(part 1 of 2)
# Autodesk Inventor assembly: #SHOOTER.3
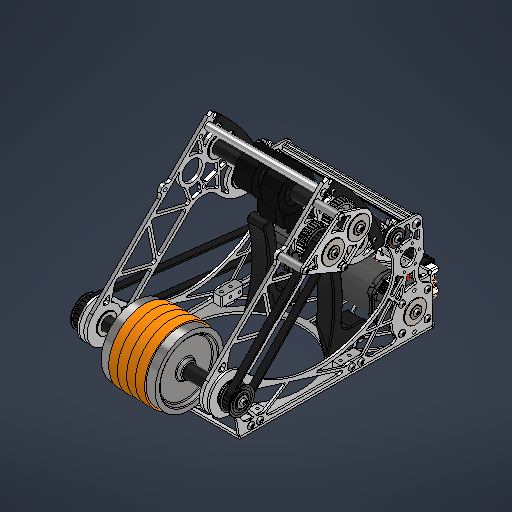
[picture p0: Inventor's stored thumbnail of the model, 512x512]
Saved by Autodesk Inventor 2026.1 (Build 301233020, 233B)
## iProperties
Created: 2026-01-27
Part Number: #SHOOTER.3
Document SubType Name: Assembly
Designer: Owen L
Mass: 4989.7 g
Surface Area: 9374.65 cm^2
Volume: 1663.66 cm^3
Density: 2.99923 g/cm^3
Author: Owen L
## Documents named in this file (57)
- C:\Users\Owen\Documents\GitHub\2026-Robot-Mechanical\Shooter\Shooter #3\#SHOOTER.3.iam
- C:\Users\Owen\Documents\GitHub\2026-Robot-Mechanical\Shooter\Shooter #3\PLATE,SHOOTER,SIDE.ipt
- C:\Users\Owen\Documents\GitHub\2026-Robot-Mechanical\#1_CAD Library\Electronics\CONTROLS,SPARK_FLEX.ipt
- C:\Users\Owen\Documents\GitHub\2026-Robot-Mechanical\#1_CAD Library\Electronics\CONTROLS,SPARK_MAX.ipt
- C:\Users\Owen\Documents\GitHub\2026-Robot-Mechanical\#1_CAD Library\Power Transmission\Bushings\PURCHASED,BUSHING,13.75mmID,0.75inOD.ipt
- C:\Users\Owen\Documents\GitHub\2026-Robot-Mechanical\#1_CAD Library\Power Transmission\Bearings\PURCHASED,HEX_BEARING.ipt
- C:\Users\Owen\Documents\GitHub\2026-Robot-Mechanical\#1_CAD Library\Motors\MOTOR,REV,NEO,VORTEX.ipt
- C:\Users\Owen\Documents\GitHub\2026-Robot-Mechanical\#1_CAD Library\Motors\MOTOR,REV,NEO,550.ipt
- C:\Users\Owen\Documents\GitHub\2026-Robot-Mechanical\#1_CAD Library\Power Transmission\UltraPlanetary\PURCHASED,REV,ULTRAPLANETARY,2-STAGE.iam
- C:\Users\Owen\Documents\GitHub\2026-Robot-Mechanical\Shooter\Shooter #3\#SHOOTER.3\Design Accelerator\PLATE,HOOD,SIDE.ipt
- C:\Users\Owen\Documents\GitHub\2026-Robot-Mechanical\Shooter\Shooter #3\#SHOOTER.3\Design Accelerator\PLATE.HOOD,PINION,GEAR.ipt
- C:\Users\Owen\Documents\GitHub\2026-Robot-Mechanical\Shooter\Shooter #3\STOCK,HEX,ROUND,HOOD.ipt
- C:\Users\Owen\Documents\GitHub\2026-Robot-Mechanical\#1_CAD Library\Power Transmission\Pulleys\PURCHASED,HTD5mm,20T,PULLEY.ipt
- C:\Users\Owen\Documents\GitHub\2026-Robot-Mechanical\Shooter\Shooter #3\STOCK,SHAFT,HEX,MOTORS.ipt
- C:\Users\Owen\Documents\GitHub\2026-Robot-Mechanical\Shooter\Shooter #3\#SHOOTER.3\Design Accelerator\PLATE,HOOD,DRIVE,GEAR,SHAFT.ipt
- C:\Users\Owen\Documents\GitHub\2026-Robot-Mechanical\Shooter\Shooter #3\#SHOOTER.3\Design Accelerator\PLATE,HOOD,DRIVE,GEAR,MOTOR.ipt
- C:\Users\Owen\Documents\GitHub\2026-Robot-Mechanical\#1_CAD Library\Power Transmission\Pulleys\PURCHASED,HTD5mm,24T,PULLEY.ipt
- C:\Users\Owen\Documents\GitHub\2026-Robot-Mechanical\Shooter\Shooter #3\STOCK,SHAFT,HEX,SHOOTER.ipt
- C:\Users\Owen\Documents\GitHub\2026-Robot-Mechanical\Shooter\Shooter #3\#SHOOTER.3\PURCHASED,10-32,0.375inOD,STANDOFF.ipt
- C:\Users\Owen\Documents\GitHub\2026-Robot-Mechanical\Shooter\Shooter #3\PLATE,BEARING,MOUNT.ipt
- C:\Users\Owen\Documents\GitHub\2026-Robot-Mechanical\Shooter\Shooter #3\STOCK,SHAFT,HEX,HOOD,WHEELS,LONG.ipt
- C:\Users\Owen\Documents\GitHub\2026-Robot-Mechanical\Shooter\Shooter #3\STOCK,SHAFT,HEX,HOOD,REVERSER.ipt
- C:\Users\Owen\Documents\GitHub\2026-Robot-Mechanical\Shooter\Shooter #3\STOCK,SHAFT,HEX,HOOD,WHEELS,SHORT.ipt
- C:\Users\Owen\Documents\GitHub\2026-Robot-Mechanical\Shooter\Shooter #3\PLATE,SHOOTER,BOTTOM.ipt
- C:\Users\Owen\Documents\GitHub\2026-Robot-Mechanical\Shooter\Shooter #3\PLATE,SHOOTER,BACK.ipt
- C:\Users\Owen\Documents\GitHub\2026-Robot-Mechanical\Shooter\Shooter #3\STOCK,CHURRO,HEX,BACK.ipt
- C:\Users\Owen\Documents\GitHub\2026-Robot-Mechanical\Shooter\Shooter #3\PURCHASED,WASHER.ipt
- C:\Users\Owen\Documents\GitHub\2026-Robot-Mechanical\#1_CAD Library\Wheels\Shooter\PURCHASED,2inOD,HEX,SHOOTER,WHEEL.ipt
- C:\Users\Owen\Documents\GitHub\2026-Robot-Mechanical\#1_CAD Library\Building Materials\Fasteners\Bolts\PURCHASED,0.25-20x0.5in,BUTTONHEAD,BOLT.ipt
- C:\Users\Owen\Documents\GitHub\2026-Robot-Mechanical\#1_CAD Library\Building Materials\Fasteners\Bolts\PURCHASED,10-32x0.5in,BUTTONHEAD,BOLT.ipt
- C:\Users\Owen\Documents\GitHub\2026-Robot-Mechanical\#1_CAD Library\Building Materials\Fasteners\Bolts\PURCHASED,M3x10mm,BUTTONHEAD,BOLT.ipt
- C:\Users\Owen\Documents\GitHub\2026-Robot-Mechanical\#1_CAD Library\Wheels\Shooter\PURCHASED,4inOD,HEX,SHOOTER,WHEEL.ipt
- C:\Users\Owen\Documents\GitHub\2026-Robot-Mechanical\Shooter\Shooter #3\3DPRINT,HOOD,DRIVEGEAR,SPACER.ipt
- C:\Users\Owen\Documents\GitHub\2026-Robot-Mechanical\Shooter\Shooter #3\3DPRINT,REVERSERGEAR,SPACER.ipt
- C:\Users\Owen\Documents\GitHub\2026-Robot-Mechanical\Shooter\Shooter #3\3DPRINT,BACKROLLERS,OPENSIDE,SPACER.ipt
- C:\Users\Owen\Documents\GitHub\2026-Robot-Mechanical\Shooter\Shooter #3\3DPRINT,BACKROLLERS,PULLEYSIDE,SPACER.ipt
- C:\Users\Owen\Documents\GitHub\2026-Robot-Mechanical\Shooter\Shooter #3\3DPRINT,BACKROLLERS,INTERROLLER,SPACER.ipt
- C:\Users\Owen\Documents\GitHub\2026-Robot-Mechanical\Shooter\Shooter #3\PLATE,FLYWHEEL.ipt
- C:\Users\Owen\Documents\GitHub\2026-Robot-Mechanical\Shooter\Shooter #3\3DPRINT,FLYWHEEL,SPACER.ipt
- C:\Users\Owen\Documents\GitHub\2026-Robot-Mechanical\#1_CAD Library\Power Transmission\Gears\PURCHASED,GEAR,20DP,30T,HEX.ipt
- C:\Users\Owen\Documents\GitHub\2026-Robot-Mechanical\Shooter\Shooter #3\3DPRINT,BACKRAIL.ipt
- C:\Users\Owen\Documents\GitHub\2026-Robot-Mechanical\Shooter\Shooter #3\3DPRINT,BACKRAIL_MIR.ipt
- C:\Users\Owen\Documents\GitHub\2026-Robot-Mechanical\Shooter\Shooter #3\PLATE,NUTBLOCK.ipt
- C:\Users\Owen\Documents\GitHub\2026-Robot-Mechanical\Shooter\Shooter #3\3DPRINT,SPARK_MAX,MOUNT.ipt
- C:\Users\Owen\Documents\GitHub\2026-Robot-Mechanical\#1_CAD Library\Building Materials\Fasteners\Bolts\PURCHASED,M4x12mm,BUTTONHEAD,BOLT.ipt
- C:\Users\Owen\Documents\GitHub\2026-Robot-Mechanical\Shooter\Shooter #3\STANDIN,130T,HTD5mm,BELT.ipt
- C:\Users\Owen\Documents\GitHub\2026-Robot-Mechanical\Shooter\Shooter #3\STANDIN,45T,HTD5mm,BELT.ipt
- C:\Users\Owen\Documents\GitHub\2026-Robot-Mechanical\Shooter\Shooter #3\STANDIN,90T,HTD5mm,BELT.ipt
- C:\Users\Owen\Documents\GitHub\2026-Robot-Mechanical\Shooter\Shooter #3\3DPRINT,FLYWHEELTOHOOD,SPACER.ipt
- C:\Users\Owen\Documents\GitHub\2026-Robot-Mechanical\Shooter\Shooter #3\STOCK,HOOD,SPACER,10-32,6.25in.ipt
- C:\Users\Owen\Documents\GitHub\2026-Robot-Mechanical\Shooter\Shooter #3\3DPRINT,SIDEPLATETOHOOD,SPACER .ipt
- C:\Users\Owen\Documents\GitHub\2026-Robot-Mechanical\Shooter\Shooter #3\3DPRINT,SIDEPLATETOHOODGEAR,SPACER.ipt
- C:\Users\Owen\Documents\GitHub\2026-Robot-Mechanical\Shooter\Shooter #3\3DPRINT,BUSHINGTOHOODDRIVEGEAR,SPACER.ipt
- C:\Users\Owen\Documents\GitHub\2026-Robot-Mechanical\Shooter\Shooter #3\PLATE,NUTBLOCK,BACK.ipt
- C:\Users\Owen\Documents\GitHub\2026-Robot-Mechanical\Shooter\Shooter #3\3DPRINT,HOOD,ALIGNMENT,PLATES.ipt
- C:\Users\Owen\Documents\GitHub\2026-Robot-Mechanical\#1_CAD Library\Building Materials\Fasteners\Bolts\PURCHASED,M3x16mm,BUTTONHEAD,BOLT.ipt
- C:\Users\Owen\Documents\GitHub\2026-Robot-Mechanical\#1_CAD Library\Building Materials\Fasteners\Nuts\PURCHASED,M3,NYLOCK,NUT.ipt
## Components (193 placed, 56 different names)
1. PLATE,SHOOTER,SIDE:1 — Insert:2, Mate:2, Insert:3, Insert:4, Mate:6, Mate:36, Insert:39, Insert:57, Insert:58, Insert:59, Insert:60, Insert:82, Insert:83, Insert:84, Insert:85, Mate:120, Insert:108, Insert:110, Insert:111, Insert:112, Insert:113, Insert:114, Insert:146, Mate:138, Mate:139
2. CONTROLS,SPARK_FLEX:1 — Mate:3, Mate:4, Mate:5, Insert:36, Insert:37
3. CONTROLS,SPARK_FLEX:2 — Mate:12, Mate:13, Mate:14, Insert:34, Insert:35
4. CONTROLS,SPARK_MAX:1 — Mate:75, Mate:135, Mate:136
5. PURCHASED,BUSHING,13.75mmID,0.75inOD:1 — Insert:3, Mate:8, Mate:166, Mate:173
6. PURCHASED,BUSHING,13.75mmID,0.75inOD:2 — Insert:7, Mate:11, Mate:170
7. PURCHASED,HEX_BEARING:1 — Insert:4, Mate:30, Mate:31, Mate:46, Mate:156
8. MOTOR,REV,NEO,VORTEX:1 — Mate:3, Mate:4, Mate:5
9. MOTOR,REV,NEO,VORTEX:2 — Mate:12, Mate:13, Mate:14
10. MOTOR,REV,NEO,550:1 — Insert:1, Mate:1
11. PURCHASED,REV,ULTRAPLANETARY,2-STAGE:1 [sub-assembly] — Insert:1, Mate:1, Insert:2, Mate:2, Flush:1, Insert:14, Mate:26
12. PLATE,HOOD,SIDE:1 — Mate:6, Mate:7, Mate:15, Insert:15, Insert:16, Mate:27, Insert:20, Mate:81, Mate:82, Symmetry:1, Insert:152, Insert:154, Insert:155, Mate:174, Insert:161, Insert:163, Insert:164, Insert:165
13. PLATE.HOOD,PINION,GEAR:1 — Mate:22, Mate:23, Mate:163, Mate:167
14. PLATE,HOOD,SIDE:2 — Mate:7, Mate:15, Insert:17, Insert:18, Mate:27, Insert:21, Insert:24, Insert:25, Insert:26, Insert:31, Insert:91, Insert:92, Insert:93, Symmetry:1, Mate:147, Mate:148, Mate:150, Insert:153, Insert:156, Insert:157, Insert:166, Insert:167, Insert:168, Insert:169
15. STOCK,HEX,ROUND,HOOD:1 — Mate:8, Flush:1, Mate:11, Mate:20, Mate:21, Mate:22, Mate:23, Mate:24, Mate:25, Insert:47, Insert:55, Mate:83, Mate:84, Mate:164, Mate:165, Mate:168, Mate:169, Mate:171, Mate:172
16. PURCHASED,HTD5mm,20T,PULLEY:1 — Mate:59, Mate:60, Mate:64, Mate:97, Mate:152
17. PLATE,SHOOTER,SIDE:2 — Insert:7, Insert:19, Mate:36, Insert:32, Insert:33, Insert:38, Insert:40, Insert:73, Insert:74, Insert:75, Insert:76, Insert:101, Insert:104, Insert:124, Insert:125, Insert:126, Insert:127, Insert:145, Mate:149
18. PURCHASED,HEX_BEARING:3 — Mate:18, Mate:19, Mate:47, Insert:39
19. PURCHASED,HEX_BEARING:4 — Insert:38
20. PLATE.HOOD,PINION,GEAR:2 — Mate:20, Mate:21, Mate:85
21. STOCK,SHAFT,HEX,MOTORS:1 — Mate:18, Mate:19, Mate:28, Mate:29, Flush:6, Insert:42, Insert:56, Rotation:1
22. PLATE,HOOD,DRIVE,GEAR,SHAFT:1 — Mate:24, Mate:25, Flush:2
23. PLATE,HOOD,DRIVE,GEAR,MOTOR:1 — Insert:14, Mate:26, Flush:2, Insert:77, Insert:78, Insert:79, Insert:80, Insert:81
24. PURCHASED,HEX_BEARING:5 — Insert:15, Mate:37, Mate:38, Flush:3
25. PURCHASED,HEX_BEARING:6 — Insert:16, Mate:39, Mate:40, Flush:4
26. PURCHASED,HEX_BEARING:7 — Insert:17, Mate:64, Mate:128
27. PURCHASED,HEX_BEARING:8 — Insert:18, Mate:63
28. PURCHASED,HTD5mm,24T,PULLEY:1 — Mate:28, Mate:29, Mate:47, Flush:6, Mate:140
29. PURCHASED,HTD5mm,24T,PULLEY:2 — Mate:32, Mate:33, Mate:46, Flush:7
30. STOCK,SHAFT,HEX,SHOOTER:1 — Mate:30, Mate:31, Mate:32, Mate:33, Flush:7, Insert:50, Insert:51, Mate:76, Mate:77, Mate:79, Mate:80, Mate:107, Mate:108, Mate:110, Mate:111, Mate:113, Mate:114, Mate:116, Mate:117, Mate:141, Mate:142, Rotation:1, Flush:9, Mate:153, Mate:154, Mate:157, Mate:158, Mate:160, Mate:161
31. PURCHASED,HEX_BEARING:9 — Insert:19, Mate:155
32. PURCHASED,HEX_BEARING:10 — Insert:20, Mate:156, Mate:162
33. PURCHASED,HEX_BEARING:11 — Insert:21, Mate:115, Mate:159
34. PURCHASED,HEX_BEARING:12 — Insert:31, Mate:41, Mate:42, Flush:5, Mate:129
35. PURCHASED,10-32,0.375inOD,STANDOFF:1 — Insert:24, Insert:97
36. PURCHASED,10-32,0.375inOD,STANDOFF:2 — Insert:25
37. PURCHASED,10-32,0.375inOD,STANDOFF:3 — Insert:26
38. PLATE,BEARING,MOUNT:1 — Insert:94, Insert:96, Insert:97, Insert:98, Insert:99, Insert:100
39. PURCHASED,HEX_BEARING:14 — Mate:88, Mate:121, Mate:122, Insert:96
40. PURCHASED,HEX_BEARING:15 — Insert:94, Mate:123
41. STOCK,SHAFT,HEX,HOOD,WHEELS,LONG:1 — Mate:37, Mate:38, Flush:3, Mate:59, Mate:60, Insert:48, Insert:53, Mate:65, Mate:66, Mate:67, Mate:68, Mate:86, Mate:87, Mate:89, Mate:90, Mate:95, Mate:96, Mate:101, Mate:102, Mate:121, Mate:122, Mate:126, Mate:127
42. STOCK,SHAFT,HEX,HOOD,REVERSER:1 — Mate:41, Mate:42, Flush:5, Insert:52, Insert:86, Mate:123, Mate:124, Mate:125, Mate:144, Mate:145
43. STOCK,SHAFT,HEX,HOOD,WHEELS,SHORT:1 — Mate:39, Mate:40, Flush:4, Mate:61, Mate:62, Insert:49, Insert:54, Mate:69, Mate:70, Mate:71, Mate:72, Mate:92, Mate:93, Mate:98, Mate:99, Mate:104, Mate:105
44. PLATE,SHOOTER,BOTTOM:1 — Mate:120, Mate:131, Insert:102, Insert:103, Insert:107, Insert:109, Insert:115, Insert:116, Insert:117, Insert:118, Insert:119, Insert:120, Insert:121, Insert:122, Insert:123, Insert:137, Insert:138, Insert:139, Insert:140, Insert:141, Insert:142, Insert:143, Insert:144, Insert:151, Mate:137, Insert:158, Mate:174, Insert:160
45. PLATE,SHOOTER,BACK:1 — Insert:32, Insert:33, Insert:34, Insert:35, Insert:36, Insert:37, Mate:75, Insert:128, Insert:129, Insert:133, Mate:134, Insert:159
46. PURCHASED,HTD5mm,20T,PULLEY:2 — Mate:61, Mate:62, Mate:63, Mate:100
47. STOCK,CHURRO,HEX,BACK:1 — Insert:40
48. PURCHASED,WASHER:1 — Insert:42, Insert:61
49. PURCHASED,2inOD,HEX,SHOOTER,WHEEL:1 — Mate:65, Mate:66, Mate:73, Mate:103
50. PURCHASED,2inOD,HEX,SHOOTER,WHEEL:2 — Mate:67, Mate:68, Mate:73, Mate:82, Flush:8, Mate:91
51. PURCHASED,2inOD,HEX,SHOOTER,WHEEL:3 — Mate:69, Mate:70, Mate:74, Mate:106
52. PURCHASED,2inOD,HEX,SHOOTER,WHEEL:4 — Mate:71, Mate:72, Mate:74, Flush:8, Mate:94
53. PURCHASED,0.25-20x0.5in,BUTTONHEAD,BOLT:1 — Insert:146
54. PURCHASED,0.25-20x0.5in,BUTTONHEAD,BOLT:4 — Insert:145
55. PURCHASED,10-32x0.5in,BUTTONHEAD,BOLT:1 — Insert:57
56. PURCHASED,M3x10mm,BUTTONHEAD,BOLT:1 — Insert:77
57. PURCHASED,WASHER:2 — Insert:47, Insert:62
58. PURCHASED,WASHER:3 — Insert:48, Insert:64
59. PURCHASED,WASHER:4 — Insert:49, Insert:63
60. PURCHASED,WASHER:5 — Insert:50, Insert:65
61. PURCHASED,WASHER:6 — Insert:51, Insert:66
62. PURCHASED,WASHER:7 — Insert:52, Insert:67
63. PURCHASED,WASHER:8 — Insert:53, Insert:68
64. PURCHASED,WASHER:9 — Insert:54, Insert:69
65. PURCHASED,WASHER:10 — Insert:55, Insert:70
66. PURCHASED,WASHER:11 — Insert:56, Insert:71
67. PURCHASED,10-32x0.5in,BUTTONHEAD,BOLT:2 — Insert:60
68. PURCHASED,10-32x0.5in,BUTTONHEAD,BOLT:3 — Insert:58
69. PURCHASED,10-32x0.5in,BUTTONHEAD,BOLT:4 — Insert:59
70. PURCHASED,10-32x0.5in,BUTTONHEAD,BOLT:5 — Insert:61
71. PURCHASED,10-32x0.5in,BUTTONHEAD,BOLT:6 — Insert:62
72. PURCHASED,10-32x0.5in,BUTTONHEAD,BOLT:7 — Insert:63
73. PURCHASED,10-32x0.5in,BUTTONHEAD,BOLT:8 — Insert:65
74. PURCHASED,10-32x0.5in,BUTTONHEAD,BOLT:9 — Insert:64
75. PURCHASED,10-32x0.5in,BUTTONHEAD,BOLT:10 — Insert:66
76. PURCHASED,10-32x0.5in,BUTTONHEAD,BOLT:11 — Insert:67
77. PURCHASED,10-32x0.5in,BUTTONHEAD,BOLT:12 — Insert:68
78. PURCHASED,10-32x0.5in,BUTTONHEAD,BOLT:13 — Insert:69
79. PURCHASED,10-32x0.5in,BUTTONHEAD,BOLT:14 — Insert:70
80. PURCHASED,10-32x0.5in,BUTTONHEAD,BOLT:15 — Insert:71
81. PURCHASED,10-32x0.5in,BUTTONHEAD,BOLT:16 — Insert:87
82. PURCHASED,10-32x0.5in,BUTTONHEAD,BOLT:17 — Insert:73
83. PURCHASED,10-32x0.5in,BUTTONHEAD,BOLT:18 — Insert:74
84. PURCHASED,10-32x0.5in,BUTTONHEAD,BOLT:19 — Insert:75
85. PURCHASED,10-32x0.5in,BUTTONHEAD,BOLT:20 — Insert:76
86. PURCHASED,M3x10mm,BUTTONHEAD,BOLT:2 — Insert:78
87. PURCHASED,M3x10mm,BUTTONHEAD,BOLT:3 — Insert:80
88. PURCHASED,M3x10mm,BUTTONHEAD,BOLT:4 — Insert:79
89. PURCHASED,M3x10mm,BUTTONHEAD,BOLT:5 — Insert:81
90. PURCHASED,M3x10mm,BUTTONHEAD,BOLT:6 — Insert:82
91. PURCHASED,M3x10mm,BUTTONHEAD,BOLT:7 — Insert:83
92. PURCHASED,M3x10mm,BUTTONHEAD,BOLT:8 — Insert:84
93. PURCHASED,M3x10mm,BUTTONHEAD,BOLT:9 — Insert:85
94. PURCHASED,4inOD,HEX,SHOOTER,WHEEL:1 — Mate:76, Mate:77, Mate:78, Mate:112
95. PURCHASED,4inOD,HEX,SHOOTER,WHEEL:2 — Mate:78, Mate:79, Mate:80, Mate:81, Mate:109
96. 3DPRINT,HOOD,DRIVEGEAR,SPACER:1 — Mate:83, Mate:84, Mate:85, Mate:163
97. 3DPRINT,REVERSERGEAR,SPACER:1 — Mate:86, Mate:87, Mate:88
98. 3DPRINT,BACKROLLERS,OPENSIDE,SPACER:1 — Mate:89, Mate:90, Mate:91
99. 3DPRINT,BACKROLLERS,OPENSIDE,SPACER:2 — Mate:92, Mate:93, Mate:94
100. 3DPRINT,BACKROLLERS,PULLEYSIDE,SPACER:1 — Mate:95, Mate:96, Mate:97
101. 3DPRINT,BACKROLLERS,PULLEYSIDE,SPACER:2 — Mate:98, Mate:99, Mate:100
102. 3DPRINT,BACKROLLERS,INTERROLLER,SPACER:1 — Mate:101, Mate:102, Mate:103
103. 3DPRINT,BACKROLLERS,INTERROLLER,SPACER:2 — Mate:104, Mate:105, Mate:106
104. PLATE,FLYWHEEL:1 — Mate:107, Mate:108, Mate:109, Mate:118, Mate:132
105. PLATE,FLYWHEEL:2 — Mate:110, Mate:111, Mate:112
106. 3DPRINT,FLYWHEEL,SPACER:1 — Mate:113, Mate:114, Mate:115
107. 3DPRINT,FLYWHEEL,SPACER:2 — Mate:116, Mate:117, Mate:118
108. PURCHASED,WASHER:12 — Insert:86, Insert:87
109. PURCHASED,10-32x0.5in,BUTTONHEAD,BOLT:21 — Insert:99
110. PURCHASED,10-32x0.5in,BUTTONHEAD,BOLT:22 — Insert:98
111. PURCHASED,10-32x0.5in,BUTTONHEAD,BOLT:23 — Insert:100
112. PURCHASED,10-32x0.5in,BUTTONHEAD,BOLT:24 — Insert:91
113. PURCHASED,10-32x0.5in,BUTTONHEAD,BOLT:25 — Insert:92
114. PURCHASED,10-32x0.5in,BUTTONHEAD,BOLT:26 — Insert:93
115. PURCHASED,GEAR,20DP,30T,HEX:1 — Mate:124, Mate:125, Mate:129, Mate:146
116. PURCHASED,GEAR,20DP,30T,HEX:2 — Mate:126, Mate:127, Mate:128
117. 3DPRINT,BACKRAIL:1 — Mate:131, Mate:132, Insert:158
118. 3DPRINT,BACKRAIL_MIR:1 — Insert:151, Mate:137
119. PLATE,NUTBLOCK:1 — Insert:101, Insert:102
120. PLATE,NUTBLOCK:2 — Insert:103, Insert:104
121. PLATE,NUTBLOCK:4 — Insert:107, Insert:108
122. PLATE,NUTBLOCK:5 — Insert:109, Insert:110
123. PURCHASED,10-32x0.5in,BUTTONHEAD,BOLT:27 — Insert:114
124. PURCHASED,10-32x0.5in,BUTTONHEAD,BOLT:28 — Insert:113
125. PURCHASED,10-32x0.5in,BUTTONHEAD,BOLT:29 — Insert:112
126. PURCHASED,10-32x0.5in,BUTTONHEAD,BOLT:30 — Insert:111
127. PURCHASED,10-32x0.5in,BUTTONHEAD,BOLT:31 — Insert:115
128. PURCHASED,10-32x0.5in,BUTTONHEAD,BOLT:32 — Insert:116
129. PURCHASED,10-32x0.5in,BUTTONHEAD,BOLT:33 — Insert:117
130. PURCHASED,10-32x0.5in,BUTTONHEAD,BOLT:34 — Insert:118
131. PURCHASED,10-32x0.5in,BUTTONHEAD,BOLT:35 — Insert:119
132. PURCHASED,10-32x0.5in,BUTTONHEAD,BOLT:36 — Insert:120
133. PURCHASED,10-32x0.5in,BUTTONHEAD,BOLT:37 — Insert:121
134. PURCHASED,10-32x0.5in,BUTTONHEAD,BOLT:38 — Insert:122
135. PURCHASED,10-32x0.5in,BUTTONHEAD,BOLT:39 — Insert:123
136. PURCHASED,10-32x0.5in,BUTTONHEAD,BOLT:40 — Insert:124
137. PURCHASED,10-32x0.5in,BUTTONHEAD,BOLT:41 — Insert:125
138. PURCHASED,10-32x0.5in,BUTTONHEAD,BOLT:42 — Insert:126
139. PURCHASED,10-32x0.5in,BUTTONHEAD,BOLT:43 — Insert:127
140. PURCHASED,10-32x0.5in,BUTTONHEAD,BOLT:44 — Insert:128
141. PURCHASED,10-32x0.5in,BUTTONHEAD,BOLT:45 — Insert:129
142. 3DPRINT,SPARK_MAX,MOUNT:1 — Insert:133, Mate:134, Mate:135, Mate:136, Insert:134, Insert:135, Insert:136
143. PURCHASED,10-32x0.5in,BUTTONHEAD,BOLT:46 — Insert:134
144. PURCHASED,10-32x0.5in,BUTTONHEAD,BOLT:47 — Insert:135
145. PURCHASED,10-32x0.5in,BUTTONHEAD,BOLT:48 — Insert:136
146. PURCHASED,M4x12mm,BUTTONHEAD,BOLT:1 — Insert:137
147. PURCHASED,M4x12mm,BUTTONHEAD,BOLT:2 — Insert:138
148. PURCHASED,M4x12mm,BUTTONHEAD,BOLT:3 — Insert:139
149. PURCHASED,M4x12mm,BUTTONHEAD,BOLT:4 — Insert:140
150. PURCHASED,M4x12mm,BUTTONHEAD,BOLT:5 — Insert:141
151. PURCHASED,M4x12mm,BUTTONHEAD,BOLT:6 — Insert:142
152. PURCHASED,M4x12mm,BUTTONHEAD,BOLT:7 — Insert:143
153. PURCHASED,M4x12mm,BUTTONHEAD,BOLT:8 — Insert:144
154. STANDIN,130T,HTD5mm,BELT:1 — Mate:138, Mate:139, Mate:140
155. PURCHASED,HTD5mm,20T,PULLEY:3 — Mate:141, Mate:142, Flush:9
156. PURCHASED,HTD5mm,20T,PULLEY:4 — Mate:144, Mate:145, Mate:146, Mate:151
157. STANDIN,45T,HTD5mm,BELT:1 — Mate:147, Mate:148, Mate:152
158. STANDIN,90T,HTD5mm,BELT:1 — Mate:149, Mate:150, Mate:151
159. 3DPRINT,FLYWHEELTOHOOD,SPACER:1 — Mate:153, Mate:154, Mate:155
160. STOCK,HOOD,SPACER,10-32,6.25in:1 — Insert:152
161. STOCK,HOOD,SPACER,10-32,6.25in:2 — Insert:153
162. PURCHASED,10-32x0.5in,BUTTONHEAD,BOLT:49 — Insert:154
163. PURCHASED,10-32x0.5in,BUTTONHEAD,BOLT:50 — Insert:156
164. PURCHASED,10-32x0.5in,BUTTONHEAD,BOLT:51 — Insert:155
165. PURCHASED,10-32x0.5in,BUTTONHEAD,BOLT:52 — Insert:157
166. 3DPRINT,SIDEPLATETOHOOD,SPACER :1 — Mate:157, Mate:158, Mate:159
167. 3DPRINT,SIDEPLATETOHOODGEAR,SPACER:1 — Mate:171, Mate:172, Mate:173
168. 3DPRINT,BUSHINGTOHOODDRIVEGEAR,SPACER:1 — Mate:164, Mate:165, Mate:166, Mate:167
169. 3DPRINT,SIDEPLATETOHOOD,SPACER :2 — Mate:160, Mate:161, Mate:162
170. 3DPRINT,BUSHINGTOHOODDRIVEGEAR,SPACER:2 — Mate:168, Mate:169, Mate:170
171. PLATE,NUTBLOCK,BACK:1 — Insert:159, Insert:160
172. 3DPRINT,HOOD,ALIGNMENT,PLATES:1 — Insert:161, Insert:165, Insert:174, Insert:175, Insert:176, Insert:177, Insert:178
173. 3DPRINT,HOOD,ALIGNMENT,PLATES:2 — Insert:163, Insert:164, Insert:179, Insert:180, Insert:181, Insert:182, Insert:183
174. 3DPRINT,HOOD,ALIGNMENT,PLATES:3 — Insert:166, Insert:167, Insert:170, Insert:171, Insert:172, Insert:173
175. 3DPRINT,HOOD,ALIGNMENT,PLATES:4 — Insert:168, Insert:169, Insert:184, Insert:185, Insert:186, Insert:187
176. PURCHASED,M3x16mm,BUTTONHEAD,BOLT:1 — Insert:170
177. PURCHASED,M3x16mm,BUTTONHEAD,BOLT:2 — Insert:171
178. PURCHASED,M3x16mm,BUTTONHEAD,BOLT:3 — Insert:172
179. PURCHASED,M3x16mm,BUTTONHEAD,BOLT:4 — Insert:173
180. PURCHASED,M3x16mm,BUTTONHEAD,BOLT:5 — Insert:174
181. PURCHASED,M3x16mm,BUTTONHEAD,BOLT:6 — Insert:175
182. PURCHASED,M3x16mm,BUTTONHEAD,BOLT:7 — Insert:176
183. PURCHASED,M3x16mm,BUTTONHEAD,BOLT:8 — Insert:177
184. PURCHASED,M3x16mm,BUTTONHEAD,BOLT:9 — Insert:178
185. PURCHASED,M3,NYLOCK,NUT:1 — Insert:186
186. PURCHASED,M3,NYLOCK,NUT:3 — Insert:187
187. PURCHASED,M3,NYLOCK,NUT:5 — Insert:185
188. PURCHASED,M3,NYLOCK,NUT:6 — Insert:184
189. PURCHASED,M3,NYLOCK,NUT:7 — Insert:183
190. PURCHASED,M3,NYLOCK,NUT:8 — Insert:182
191. PURCHASED,M3,NYLOCK,NUT:9 — Insert:181
192. PURCHASED,M3,NYLOCK,NUT:10 — Insert:180
193. PURCHASED,M3,NYLOCK,NUT:11 — Insert:179
## Relationships (314: Insert 153, Mate 150, Flush 9, Symmetry 1, RelateRotation 1)
- Insert:1: MOTOR,REV,NEO,550:1 ↔ PURCHASED,REV,ULTRAPLANETARY,2-STAGE:1
- Mate:1: MOTOR,REV,NEO,550:1 ↔ PURCHASED,REV,ULTRAPLANETARY,2-STAGE:1
- Insert:2: PLATE,SHOOTER,SIDE:1 ↔ PURCHASED,REV,ULTRAPLANETARY,2-STAGE:1
- Mate:2: PLATE,SHOOTER,SIDE:1 ↔ PURCHASED,REV,ULTRAPLANETARY,2-STAGE:1
- Insert:3: PLATE,SHOOTER,SIDE:1 ↔ PURCHASED,BUSHING,13.75mmID,0.75inOD:1
- Insert:4: PLATE,SHOOTER,SIDE:1 ↔ PURCHASED,HEX_BEARING:1
- Mate:3: CONTROLS,SPARK_FLEX:1 ↔ MOTOR,REV,NEO,VORTEX:1
- Mate:4: CONTROLS,SPARK_FLEX:1 ↔ MOTOR,REV,NEO,VORTEX:1
- Mate:5: CONTROLS,SPARK_FLEX:1 ↔ MOTOR,REV,NEO,VORTEX:1
- Mate:6: PLATE,SHOOTER,SIDE:1 ↔ PLATE,HOOD,SIDE:1
- Mate:7 (158.75 mm): PLATE,HOOD,SIDE:1 ↔ PLATE,HOOD,SIDE:2
- Mate:8: PURCHASED,BUSHING,13.75mmID,0.75inOD:1 ↔ STOCK,HEX,ROUND,HOOD:1
- Flush:1 (-6.35 mm): PURCHASED,REV,ULTRAPLANETARY,2-STAGE:1 ↔ STOCK,HEX,ROUND,HOOD:1
- Insert:7: PURCHASED,BUSHING,13.75mmID,0.75inOD:2 ↔ PLATE,SHOOTER,SIDE:2
- Mate:11: PURCHASED,BUSHING,13.75mmID,0.75inOD:2 ↔ STOCK,HEX,ROUND,HOOD:1
- Mate:12: CONTROLS,SPARK_FLEX:2 ↔ MOTOR,REV,NEO,VORTEX:2
- Mate:13: CONTROLS,SPARK_FLEX:2 ↔ MOTOR,REV,NEO,VORTEX:2
- Mate:14: CONTROLS,SPARK_FLEX:2 ↔ MOTOR,REV,NEO,VORTEX:2
- Mate:15: PLATE,HOOD,SIDE:1 ↔ PLATE,HOOD,SIDE:2
- Mate:18: PURCHASED,HEX_BEARING:3 ↔ STOCK,SHAFT,HEX,MOTORS:1
- Mate:19: PURCHASED,HEX_BEARING:3 ↔ STOCK,SHAFT,HEX,MOTORS:1
- Mate:20: STOCK,HEX,ROUND,HOOD:1 ↔ PLATE.HOOD,PINION,GEAR:2
- Mate:21: STOCK,HEX,ROUND,HOOD:1 ↔ PLATE.HOOD,PINION,GEAR:2
- Mate:22: PLATE.HOOD,PINION,GEAR:1 ↔ STOCK,HEX,ROUND,HOOD:1
- Mate:23: PLATE.HOOD,PINION,GEAR:1 ↔ STOCK,HEX,ROUND,HOOD:1
- Mate:24: STOCK,HEX,ROUND,HOOD:1 ↔ PLATE,HOOD,DRIVE,GEAR,SHAFT:1
- Mate:25: STOCK,HEX,ROUND,HOOD:1 ↔ PLATE,HOOD,DRIVE,GEAR,SHAFT:1
- Insert:14: PURCHASED,REV,ULTRAPLANETARY,2-STAGE:1 ↔ PLATE,HOOD,DRIVE,GEAR,MOTOR:1
- Mate:26: PURCHASED,REV,ULTRAPLANETARY,2-STAGE:1 ↔ PLATE,HOOD,DRIVE,GEAR,MOTOR:1
- Flush:2: PLATE,HOOD,DRIVE,GEAR,SHAFT:1 ↔ PLATE,HOOD,DRIVE,GEAR,MOTOR:1
- Insert:15: PLATE,HOOD,SIDE:1 ↔ PURCHASED,HEX_BEARING:5
- Insert:16: PLATE,HOOD,SIDE:1 ↔ PURCHASED,HEX_BEARING:6
- Insert:17: PLATE,HOOD,SIDE:2 ↔ PURCHASED,HEX_BEARING:7
- Insert:18: PLATE,HOOD,SIDE:2 ↔ PURCHASED,HEX_BEARING:8
- Mate:27: PLATE,HOOD,SIDE:1 ↔ PLATE,HOOD,SIDE:2
- Mate:28: STOCK,SHAFT,HEX,MOTORS:1 ↔ PURCHASED,HTD5mm,24T,PULLEY:1
- Mate:29: STOCK,SHAFT,HEX,MOTORS:1 ↔ PURCHASED,HTD5mm,24T,PULLEY:1
- Mate:30: PURCHASED,HEX_BEARING:1 ↔ STOCK,SHAFT,HEX,SHOOTER:1
- Mate:31: PURCHASED,HEX_BEARING:1 ↔ STOCK,SHAFT,HEX,SHOOTER:1
- Insert:19: PLATE,SHOOTER,SIDE:2 ↔ PURCHASED,HEX_BEARING:9
- Insert:20: PLATE,HOOD,SIDE:1 ↔ PURCHASED,HEX_BEARING:10
- Insert:21: PLATE,HOOD,SIDE:2 ↔ PURCHASED,HEX_BEARING:11
- Mate:32: PURCHASED,HTD5mm,24T,PULLEY:2 ↔ STOCK,SHAFT,HEX,SHOOTER:1
- Mate:33: PURCHASED,HTD5mm,24T,PULLEY:2 ↔ STOCK,SHAFT,HEX,SHOOTER:1
- Mate:36: PLATE,SHOOTER,SIDE:1 ↔ PLATE,SHOOTER,SIDE:2
- Insert:24: PLATE,HOOD,SIDE:2 ↔ PURCHASED,10-32,0.375inOD,STANDOFF:1
- Insert:25: PLATE,HOOD,SIDE:2 ↔ PURCHASED,10-32,0.375inOD,STANDOFF:2
- Insert:26: PLATE,HOOD,SIDE:2 ↔ PURCHASED,10-32,0.375inOD,STANDOFF:3
- Mate:37: PURCHASED,HEX_BEARING:5 ↔ STOCK,SHAFT,HEX,HOOD,WHEELS,LONG:1
- Mate:38: PURCHASED,HEX_BEARING:5 ↔ STOCK,SHAFT,HEX,HOOD,WHEELS,LONG:1
- Flush:3: PURCHASED,HEX_BEARING:5 ↔ STOCK,SHAFT,HEX,HOOD,WHEELS,LONG:1
- Insert:31: PLATE,HOOD,SIDE:2 ↔ PURCHASED,HEX_BEARING:12
- Mate:39: PURCHASED,HEX_BEARING:6 ↔ STOCK,SHAFT,HEX,HOOD,WHEELS,SHORT:1
- Mate:40: PURCHASED,HEX_BEARING:6 ↔ STOCK,SHAFT,HEX,HOOD,WHEELS,SHORT:1
- Flush:4: PURCHASED,HEX_BEARING:6 ↔ STOCK,SHAFT,HEX,HOOD,WHEELS,SHORT:1
- Mate:41: PURCHASED,HEX_BEARING:12 ↔ STOCK,SHAFT,HEX,HOOD,REVERSER:1
- Mate:42: PURCHASED,HEX_BEARING:12 ↔ STOCK,SHAFT,HEX,HOOD,REVERSER:1
- Flush:5: PURCHASED,HEX_BEARING:12 ↔ STOCK,SHAFT,HEX,HOOD,REVERSER:1
- Mate:46: PURCHASED,HEX_BEARING:1 ↔ PURCHASED,HTD5mm,24T,PULLEY:2
- Mate:47: PURCHASED,HEX_BEARING:3 ↔ PURCHASED,HTD5mm,24T,PULLEY:1
- Mate:59: PURCHASED,HTD5mm,20T,PULLEY:1 ↔ STOCK,SHAFT,HEX,HOOD,WHEELS,LONG:1
- Mate:60: PURCHASED,HTD5mm,20T,PULLEY:1 ↔ STOCK,SHAFT,HEX,HOOD,WHEELS,LONG:1
- Mate:61: STOCK,SHAFT,HEX,HOOD,WHEELS,SHORT:1 ↔ PURCHASED,HTD5mm,20T,PULLEY:2
- Mate:62: STOCK,SHAFT,HEX,HOOD,WHEELS,SHORT:1 ↔ PURCHASED,HTD5mm,20T,PULLEY:2
- Mate:63: PURCHASED,HEX_BEARING:8 ↔ PURCHASED,HTD5mm,20T,PULLEY:2
- Mate:64: PURCHASED,HTD5mm,20T,PULLEY:1 ↔ PURCHASED,HEX_BEARING:7
- Insert:32: PLATE,SHOOTER,SIDE:2 ↔ PLATE,SHOOTER,BACK:1
- Insert:33: PLATE,SHOOTER,SIDE:2 ↔ PLATE,SHOOTER,BACK:1
- Insert:34: CONTROLS,SPARK_FLEX:2 ↔ PLATE,SHOOTER,BACK:1
- Insert:35: CONTROLS,SPARK_FLEX:2 ↔ PLATE,SHOOTER,BACK:1
- Insert:36: CONTROLS,SPARK_FLEX:1 ↔ PLATE,SHOOTER,BACK:1
- Insert:37: CONTROLS,SPARK_FLEX:1 ↔ PLATE,SHOOTER,BACK:1
- Insert:38: PLATE,SHOOTER,SIDE:2 ↔ PURCHASED,HEX_BEARING:4
- Insert:39: PLATE,SHOOTER,SIDE:1 ↔ PURCHASED,HEX_BEARING:3
- Flush:6: STOCK,SHAFT,HEX,MOTORS:1 ↔ PURCHASED,HTD5mm,24T,PULLEY:1
- Flush:7: PURCHASED,HTD5mm,24T,PULLEY:2 ↔ STOCK,SHAFT,HEX,SHOOTER:1
- Insert:40: PLATE,SHOOTER,SIDE:2 ↔ STOCK,CHURRO,HEX,BACK:1
- Insert:42: STOCK,SHAFT,HEX,MOTORS:1 ↔ PURCHASED,WASHER:1
- Insert:47: STOCK,HEX,ROUND,HOOD:1 ↔ PURCHASED,WASHER:2
- Insert:48: STOCK,SHAFT,HEX,HOOD,WHEELS,LONG:1 ↔ PURCHASED,WASHER:3
- Insert:49: STOCK,SHAFT,HEX,HOOD,WHEELS,SHORT:1 ↔ PURCHASED,WASHER:4
- Insert:50: STOCK,SHAFT,HEX,SHOOTER:1 ↔ PURCHASED,WASHER:5
- Insert:51: STOCK,SHAFT,HEX,SHOOTER:1 ↔ PURCHASED,WASHER:6
- Insert:52: STOCK,SHAFT,HEX,HOOD,REVERSER:1 ↔ PURCHASED,WASHER:7
- Insert:53: STOCK,SHAFT,HEX,HOOD,WHEELS,LONG:1 ↔ PURCHASED,WASHER:8
- Insert:54: STOCK,SHAFT,HEX,HOOD,WHEELS,SHORT:1 ↔ PURCHASED,WASHER:9
- Insert:55: STOCK,HEX,ROUND,HOOD:1 ↔ PURCHASED,WASHER:10
- Insert:56: STOCK,SHAFT,HEX,MOTORS:1 ↔ PURCHASED,WASHER:11
- Mate:65: STOCK,SHAFT,HEX,HOOD,WHEELS,LONG:1 ↔ PURCHASED,2inOD,HEX,SHOOTER,WHEEL:1
- Mate:66: STOCK,SHAFT,HEX,HOOD,WHEELS,LONG:1 ↔ PURCHASED,2inOD,HEX,SHOOTER,WHEEL:1
- Mate:67: STOCK,SHAFT,HEX,HOOD,WHEELS,LONG:1 ↔ PURCHASED,2inOD,HEX,SHOOTER,WHEEL:2
- Mate:68: STOCK,SHAFT,HEX,HOOD,WHEELS,LONG:1 ↔ PURCHASED,2inOD,HEX,SHOOTER,WHEEL:2
- Mate:69: STOCK,SHAFT,HEX,HOOD,WHEELS,SHORT:1 ↔ PURCHASED,2inOD,HEX,SHOOTER,WHEEL:3
- Mate:70: STOCK,SHAFT,HEX,HOOD,WHEELS,SHORT:1 ↔ PURCHASED,2inOD,HEX,SHOOTER,WHEEL:3
- Mate:71: STOCK,SHAFT,HEX,HOOD,WHEELS,SHORT:1 ↔ PURCHASED,2inOD,HEX,SHOOTER,WHEEL:4
- Mate:72: STOCK,SHAFT,HEX,HOOD,WHEELS,SHORT:1 ↔ PURCHASED,2inOD,HEX,SHOOTER,WHEEL:4
- Mate:73 (12.7 mm): PURCHASED,2inOD,HEX,SHOOTER,WHEEL:1 ↔ PURCHASED,2inOD,HEX,SHOOTER,WHEEL:2
- Mate:74 (12.7 mm): PURCHASED,2inOD,HEX,SHOOTER,WHEEL:3 ↔ PURCHASED,2inOD,HEX,SHOOTER,WHEEL:4
- Insert:57: PLATE,SHOOTER,SIDE:1 ↔ PURCHASED,10-32x0.5in,BUTTONHEAD,BOLT:1
- Insert:58: PLATE,SHOOTER,SIDE:1 ↔ PURCHASED,10-32x0.5in,BUTTONHEAD,BOLT:3
- Insert:59: PLATE,SHOOTER,SIDE:1 ↔ PURCHASED,10-32x0.5in,BUTTONHEAD,BOLT:4
- Insert:60: PLATE,SHOOTER,SIDE:1 ↔ PURCHASED,10-32x0.5in,BUTTONHEAD,BOLT:2
- Insert:61: PURCHASED,WASHER:1 ↔ PURCHASED,10-32x0.5in,BUTTONHEAD,BOLT:5
- Insert:62: PURCHASED,WASHER:2 ↔ PURCHASED,10-32x0.5in,BUTTONHEAD,BOLT:6
- Insert:63: PURCHASED,WASHER:4 ↔ PURCHASED,10-32x0.5in,BUTTONHEAD,BOLT:7
- Insert:64: PURCHASED,WASHER:3 ↔ PURCHASED,10-32x0.5in,BUTTONHEAD,BOLT:9
- Insert:65: PURCHASED,WASHER:5 ↔ PURCHASED,10-32x0.5in,BUTTONHEAD,BOLT:8
- Insert:66: PURCHASED,WASHER:6 ↔ PURCHASED,10-32x0.5in,BUTTONHEAD,BOLT:10
- Insert:67: PURCHASED,WASHER:7 ↔ PURCHASED,10-32x0.5in,BUTTONHEAD,BOLT:11
- Insert:68: PURCHASED,WASHER:8 ↔ PURCHASED,10-32x0.5in,BUTTONHEAD,BOLT:12
- Insert:69: PURCHASED,WASHER:9 ↔ PURCHASED,10-32x0.5in,BUTTONHEAD,BOLT:13
- Insert:70: PURCHASED,WASHER:10 ↔ PURCHASED,10-32x0.5in,BUTTONHEAD,BOLT:14
- Insert:71: PURCHASED,WASHER:11 ↔ PURCHASED,10-32x0.5in,BUTTONHEAD,BOLT:15
- Insert:73: PLATE,SHOOTER,SIDE:2 ↔ PURCHASED,10-32x0.5in,BUTTONHEAD,BOLT:17
- Insert:74: PLATE,SHOOTER,SIDE:2 ↔ PURCHASED,10-32x0.5in,BUTTONHEAD,BOLT:18
- Insert:75: PLATE,SHOOTER,SIDE:2 ↔ PURCHASED,10-32x0.5in,BUTTONHEAD,BOLT:19
- Insert:76: PLATE,SHOOTER,SIDE:2 ↔ PURCHASED,10-32x0.5in,BUTTONHEAD,BOLT:20
- Insert:77: PLATE,HOOD,DRIVE,GEAR,MOTOR:1 ↔ PURCHASED,M3x10mm,BUTTONHEAD,BOLT:1
- Insert:78: PLATE,HOOD,DRIVE,GEAR,MOTOR:1 ↔ PURCHASED,M3x10mm,BUTTONHEAD,BOLT:2
- Insert:79: PLATE,HOOD,DRIVE,GEAR,MOTOR:1 ↔ PURCHASED,M3x10mm,BUTTONHEAD,BOLT:4
- Insert:80: PLATE,HOOD,DRIVE,GEAR,MOTOR:1 ↔ PURCHASED,M3x10mm,BUTTONHEAD,BOLT:3
- Insert:81: PLATE,HOOD,DRIVE,GEAR,MOTOR:1 ↔ PURCHASED,M3x10mm,BUTTONHEAD,BOLT:5
- Insert:82: PLATE,SHOOTER,SIDE:1 ↔ PURCHASED,M3x10mm,BUTTONHEAD,BOLT:6
- Insert:83: PLATE,SHOOTER,SIDE:1 ↔ PURCHASED,M3x10mm,BUTTONHEAD,BOLT:7
- Insert:84: PLATE,SHOOTER,SIDE:1 ↔ PURCHASED,M3x10mm,BUTTONHEAD,BOLT:8
- Insert:85: PLATE,SHOOTER,SIDE:1 ↔ PURCHASED,M3x10mm,BUTTONHEAD,BOLT:9
- Mate:75: CONTROLS,SPARK_MAX:1 ↔ PLATE,SHOOTER,BACK:1
- Mate:76: STOCK,SHAFT,HEX,SHOOTER:1 ↔ PURCHASED,4inOD,HEX,SHOOTER,WHEEL:1
- Mate:77: STOCK,SHAFT,HEX,SHOOTER:1 ↔ PURCHASED,4inOD,HEX,SHOOTER,WHEEL:1
- Mate:78: PURCHASED,4inOD,HEX,SHOOTER,WHEEL:1 ↔ PURCHASED,4inOD,HEX,SHOOTER,WHEEL:2
- Mate:79: STOCK,SHAFT,HEX,SHOOTER:1 ↔ PURCHASED,4inOD,HEX,SHOOTER,WHEEL:2
- Mate:80: STOCK,SHAFT,HEX,SHOOTER:1 ↔ PURCHASED,4inOD,HEX,SHOOTER,WHEEL:2
- Mate:81 (53.975 mm): PLATE,HOOD,SIDE:1 ↔ PURCHASED,4inOD,HEX,SHOOTER,WHEEL:2
- Mate:82 (47.625 mm): PLATE,HOOD,SIDE:1 ↔ PURCHASED,2inOD,HEX,SHOOTER,WHEEL:2
- Flush:8: PURCHASED,2inOD,HEX,SHOOTER,WHEEL:2 ↔ PURCHASED,2inOD,HEX,SHOOTER,WHEEL:4
- Mate:83: STOCK,HEX,ROUND,HOOD:1 ↔ 3DPRINT,HOOD,DRIVEGEAR,SPACER:1
- Mate:84: STOCK,HEX,ROUND,HOOD:1 ↔ 3DPRINT,HOOD,DRIVEGEAR,SPACER:1
- Mate:85: PLATE.HOOD,PINION,GEAR:2 ↔ 3DPRINT,HOOD,DRIVEGEAR,SPACER:1
- Mate:86: STOCK,SHAFT,HEX,HOOD,WHEELS,LONG:1 ↔ 3DPRINT,REVERSERGEAR,SPACER:1
- Mate:87: STOCK,SHAFT,HEX,HOOD,WHEELS,LONG:1 ↔ 3DPRINT,REVERSERGEAR,SPACER:1
- Mate:88: PURCHASED,HEX_BEARING:14 ↔ 3DPRINT,REVERSERGEAR,SPACER:1
- Mate:89: STOCK,SHAFT,HEX,HOOD,WHEELS,LONG:1 ↔ 3DPRINT,BACKROLLERS,OPENSIDE,SPACER:1
- Mate:90: STOCK,SHAFT,HEX,HOOD,WHEELS,LONG:1 ↔ 3DPRINT,BACKROLLERS,OPENSIDE,SPACER:1
- Mate:91: PURCHASED,2inOD,HEX,SHOOTER,WHEEL:2 ↔ 3DPRINT,BACKROLLERS,OPENSIDE,SPACER:1
- Mate:92: STOCK,SHAFT,HEX,HOOD,WHEELS,SHORT:1 ↔ 3DPRINT,BACKROLLERS,OPENSIDE,SPACER:2
- Mate:93: STOCK,SHAFT,HEX,HOOD,WHEELS,SHORT:1 ↔ 3DPRINT,BACKROLLERS,OPENSIDE,SPACER:2
- Mate:94: PURCHASED,2inOD,HEX,SHOOTER,WHEEL:4 ↔ 3DPRINT,BACKROLLERS,OPENSIDE,SPACER:2
- Mate:95: STOCK,SHAFT,HEX,HOOD,WHEELS,LONG:1 ↔ 3DPRINT,BACKROLLERS,PULLEYSIDE,SPACER:1
- Mate:96: STOCK,SHAFT,HEX,HOOD,WHEELS,LONG:1 ↔ 3DPRINT,BACKROLLERS,PULLEYSIDE,SPACER:1
- Mate:97: PURCHASED,HTD5mm,20T,PULLEY:1 ↔ 3DPRINT,BACKROLLERS,PULLEYSIDE,SPACER:1
- Mate:98: STOCK,SHAFT,HEX,HOOD,WHEELS,SHORT:1 ↔ 3DPRINT,BACKROLLERS,PULLEYSIDE,SPACER:2
- Mate:99: STOCK,SHAFT,HEX,HOOD,WHEELS,SHORT:1 ↔ 3DPRINT,BACKROLLERS,PULLEYSIDE,SPACER:2
- Mate:100: PURCHASED,HTD5mm,20T,PULLEY:2 ↔ 3DPRINT,BACKROLLERS,PULLEYSIDE,SPACER:2
- Mate:101: STOCK,SHAFT,HEX,HOOD,WHEELS,LONG:1 ↔ 3DPRINT,BACKROLLERS,INTERROLLER,SPACER:1
- Mate:102: STOCK,SHAFT,HEX,HOOD,WHEELS,LONG:1 ↔ 3DPRINT,BACKROLLERS,INTERROLLER,SPACER:1
- Mate:103: PURCHASED,2inOD,HEX,SHOOTER,WHEEL:1 ↔ 3DPRINT,BACKROLLERS,INTERROLLER,SPACER:1
- Mate:104: STOCK,SHAFT,HEX,HOOD,WHEELS,SHORT:1 ↔ 3DPRINT,BACKROLLERS,INTERROLLER,SPACER:2
- Mate:105: STOCK,SHAFT,HEX,HOOD,WHEELS,SHORT:1 ↔ 3DPRINT,BACKROLLERS,INTERROLLER,SPACER:2
- Mate:106: PURCHASED,2inOD,HEX,SHOOTER,WHEEL:3 ↔ 3DPRINT,BACKROLLERS,INTERROLLER,SPACER:2
- Mate:107: STOCK,SHAFT,HEX,SHOOTER:1 ↔ PLATE,FLYWHEEL:1
- Mate:108: STOCK,SHAFT,HEX,SHOOTER:1 ↔ PLATE,FLYWHEEL:1
- Mate:109: PURCHASED,4inOD,HEX,SHOOTER,WHEEL:2 ↔ PLATE,FLYWHEEL:1
- Mate:110: STOCK,SHAFT,HEX,SHOOTER:1 ↔ PLATE,FLYWHEEL:2
- Mate:111: STOCK,SHAFT,HEX,SHOOTER:1 ↔ PLATE,FLYWHEEL:2
- Mate:112: PURCHASED,4inOD,HEX,SHOOTER,WHEEL:1 ↔ PLATE,FLYWHEEL:2
- Mate:113: STOCK,SHAFT,HEX,SHOOTER:1 ↔ 3DPRINT,FLYWHEEL,SPACER:1
- Mate:114: STOCK,SHAFT,HEX,SHOOTER:1 ↔ 3DPRINT,FLYWHEEL,SPACER:1
- Mate:115: PURCHASED,HEX_BEARING:11 ↔ 3DPRINT,FLYWHEEL,SPACER:1
- Mate:116: STOCK,SHAFT,HEX,SHOOTER:1 ↔ 3DPRINT,FLYWHEEL,SPACER:2
- Mate:117: STOCK,SHAFT,HEX,SHOOTER:1 ↔ 3DPRINT,FLYWHEEL,SPACER:2
- Mate:118: PLATE,FLYWHEEL:1 ↔ 3DPRINT,FLYWHEEL,SPACER:2
- Insert:86: STOCK,SHAFT,HEX,HOOD,REVERSER:1 ↔ PURCHASED,WASHER:12
- Insert:87: PURCHASED,10-32x0.5in,BUTTONHEAD,BOLT:16 ↔ PURCHASED,WASHER:12
- Insert:91: PLATE,HOOD,SIDE:2 ↔ PURCHASED,10-32x0.5in,BUTTONHEAD,BOLT:24
- Insert:92: PLATE,HOOD,SIDE:2 ↔ PURCHASED,10-32x0.5in,BUTTONHEAD,BOLT:25
- Insert:93: PLATE,HOOD,SIDE:2 ↔ PURCHASED,10-32x0.5in,BUTTONHEAD,BOLT:26
- Mate:120: PLATE,SHOOTER,SIDE:1 ↔ PLATE,SHOOTER,BOTTOM:1
- Mate:121: PURCHASED,HEX_BEARING:14 ↔ STOCK,SHAFT,HEX,HOOD,WHEELS,LONG:1
- Mate:122: PURCHASED,HEX_BEARING:14 ↔ STOCK,SHAFT,HEX,HOOD,WHEELS,LONG:1
- Insert:94: PLATE,BEARING,MOUNT:1 ↔ PURCHASED,HEX_BEARING:15
- Insert:96: PLATE,BEARING,MOUNT:1 ↔ PURCHASED,HEX_BEARING:14
- Mate:123: PURCHASED,HEX_BEARING:15 ↔ STOCK,SHAFT,HEX,HOOD,REVERSER:1
- Insert:97: PURCHASED,10-32,0.375inOD,STANDOFF:1 ↔ PLATE,BEARING,MOUNT:1
- Insert:98: PLATE,BEARING,MOUNT:1 ↔ PURCHASED,10-32x0.5in,BUTTONHEAD,BOLT:22
- Insert:99: PLATE,BEARING,MOUNT:1 ↔ PURCHASED,10-32x0.5in,BUTTONHEAD,BOLT:21
- Insert:100: PLATE,BEARING,MOUNT:1 ↔ PURCHASED,10-32x0.5in,BUTTONHEAD,BOLT:23
- Mate:124: STOCK,SHAFT,HEX,HOOD,REVERSER:1 ↔ PURCHASED,GEAR,20DP,30T,HEX:1
- Mate:125: STOCK,SHAFT,HEX,HOOD,REVERSER:1 ↔ PURCHASED,GEAR,20DP,30T,HEX:1
- Mate:126: STOCK,SHAFT,HEX,HOOD,WHEELS,LONG:1 ↔ PURCHASED,GEAR,20DP,30T,HEX:2
- Mate:127: STOCK,SHAFT,HEX,HOOD,WHEELS,LONG:1 ↔ PURCHASED,GEAR,20DP,30T,HEX:2
- Mate:128: PURCHASED,HEX_BEARING:7 ↔ PURCHASED,GEAR,20DP,30T,HEX:2
- Mate:129: PURCHASED,HEX_BEARING:12 ↔ PURCHASED,GEAR,20DP,30T,HEX:1
- Mate:131: PLATE,SHOOTER,BOTTOM:1 ↔ 3DPRINT,BACKRAIL:1
- Mate:132: PLATE,FLYWHEEL:1 ↔ 3DPRINT,BACKRAIL:1
- Symmetry:1: PLATE,HOOD,SIDE:1 ↔ PLATE,HOOD,SIDE:2
- Insert:101: PLATE,SHOOTER,SIDE:2 ↔ PLATE,NUTBLOCK:1
- Insert:102: PLATE,SHOOTER,BOTTOM:1 ↔ PLATE,NUTBLOCK:1
- Insert:103: PLATE,SHOOTER,BOTTOM:1 ↔ PLATE,NUTBLOCK:2
- Insert:104: PLATE,SHOOTER,SIDE:2 ↔ PLATE,NUTBLOCK:2
- Insert:107: PLATE,SHOOTER,BOTTOM:1 ↔ PLATE,NUTBLOCK:4
- Insert:108: PLATE,SHOOTER,SIDE:1 ↔ PLATE,NUTBLOCK:4
- Insert:109: PLATE,SHOOTER,BOTTOM:1 ↔ PLATE,NUTBLOCK:5
- Insert:110: PLATE,SHOOTER,SIDE:1 ↔ PLATE,NUTBLOCK:5
- Insert:111: PLATE,SHOOTER,SIDE:1 ↔ PURCHASED,10-32x0.5in,BUTTONHEAD,BOLT:30
- Insert:112: PLATE,SHOOTER,SIDE:1 ↔ PURCHASED,10-32x0.5in,BUTTONHEAD,BOLT:29
- Insert:113: PLATE,SHOOTER,SIDE:1 ↔ PURCHASED,10-32x0.5in,BUTTONHEAD,BOLT:28
- Insert:114: PLATE,SHOOTER,SIDE:1 ↔ PURCHASED,10-32x0.5in,BUTTONHEAD,BOLT:27
- Insert:115: PLATE,SHOOTER,BOTTOM:1 ↔ PURCHASED,10-32x0.5in,BUTTONHEAD,BOLT:31
- Insert:116: PLATE,SHOOTER,BOTTOM:1 ↔ PURCHASED,10-32x0.5in,BUTTONHEAD,BOLT:32
- Insert:117: PLATE,SHOOTER,BOTTOM:1 ↔ PURCHASED,10-32x0.5in,BUTTONHEAD,BOLT:33
- Insert:118: PLATE,SHOOTER,BOTTOM:1 ↔ PURCHASED,10-32x0.5in,BUTTONHEAD,BOLT:34
- Insert:119: PLATE,SHOOTER,BOTTOM:1 ↔ PURCHASED,10-32x0.5in,BUTTONHEAD,BOLT:35
- Insert:120: PLATE,SHOOTER,BOTTOM:1 ↔ PURCHASED,10-32x0.5in,BUTTONHEAD,BOLT:36
- Insert:121: PLATE,SHOOTER,BOTTOM:1 ↔ PURCHASED,10-32x0.5in,BUTTONHEAD,BOLT:37
- Insert:122: PLATE,SHOOTER,BOTTOM:1 ↔ PURCHASED,10-32x0.5in,BUTTONHEAD,BOLT:38
- Insert:123: PLATE,SHOOTER,BOTTOM:1 ↔ PURCHASED,10-32x0.5in,BUTTONHEAD,BOLT:39
- Insert:124: PLATE,SHOOTER,SIDE:2 ↔ PURCHASED,10-32x0.5in,BUTTONHEAD,BOLT:40
- Insert:125: PLATE,SHOOTER,SIDE:2 ↔ PURCHASED,10-32x0.5in,BUTTONHEAD,BOLT:41
- Insert:126: PLATE,SHOOTER,SIDE:2 ↔ PURCHASED,10-32x0.5in,BUTTONHEAD,BOLT:42
- Insert:127: PLATE,SHOOTER,SIDE:2 ↔ PURCHASED,10-32x0.5in,BUTTONHEAD,BOLT:43
- Insert:128: PLATE,SHOOTER,BACK:1 ↔ PURCHASED,10-32x0.5in,BUTTONHEAD,BOLT:44
- Insert:129: PLATE,SHOOTER,BACK:1 ↔ PURCHASED,10-32x0.5in,BUTTONHEAD,BOLT:45
- Insert:133: PLATE,SHOOTER,BACK:1 ↔ 3DPRINT,SPARK_MAX,MOUNT:1
- Mate:134: PLATE,SHOOTER,BACK:1 ↔ 3DPRINT,SPARK_MAX,MOUNT:1
- Mate:135 (0.762 mm): CONTROLS,SPARK_MAX:1 ↔ 3DPRINT,SPARK_MAX,MOUNT:1
- Mate:136 (11.938 mm): CONTROLS,SPARK_MAX:1 ↔ 3DPRINT,SPARK_MAX,MOUNT:1
- Insert:134: 3DPRINT,SPARK_MAX,MOUNT:1 ↔ PURCHASED,10-32x0.5in,BUTTONHEAD,BOLT:46
- Insert:135: 3DPRINT,SPARK_MAX,MOUNT:1 ↔ PURCHASED,10-32x0.5in,BUTTONHEAD,BOLT:47
- Insert:136: 3DPRINT,SPARK_MAX,MOUNT:1 ↔ PURCHASED,10-32x0.5in,BUTTONHEAD,BOLT:48
- Insert:137: PLATE,SHOOTER,BOTTOM:1 ↔ PURCHASED,M4x12mm,BUTTONHEAD,BOLT:1
- Insert:138: PLATE,SHOOTER,BOTTOM:1 ↔ PURCHASED,M4x12mm,BUTTONHEAD,BOLT:2
- Insert:139: PLATE,SHOOTER,BOTTOM:1 ↔ PURCHASED,M4x12mm,BUTTONHEAD,BOLT:3
- Insert:140: PLATE,SHOOTER,BOTTOM:1 ↔ PURCHASED,M4x12mm,BUTTONHEAD,BOLT:4
- Insert:141: PLATE,SHOOTER,BOTTOM:1 ↔ PURCHASED,M4x12mm,BUTTONHEAD,BOLT:5
- Insert:142: PLATE,SHOOTER,BOTTOM:1 ↔ PURCHASED,M4x12mm,BUTTONHEAD,BOLT:6
- Insert:143: PLATE,SHOOTER,BOTTOM:1 ↔ PURCHASED,M4x12mm,BUTTONHEAD,BOLT:7
- Insert:144: PLATE,SHOOTER,BOTTOM:1 ↔ PURCHASED,M4x12mm,BUTTONHEAD,BOLT:8